# Autodesk Inventor assembly: Bed Arm Back for 4040 - Assembly
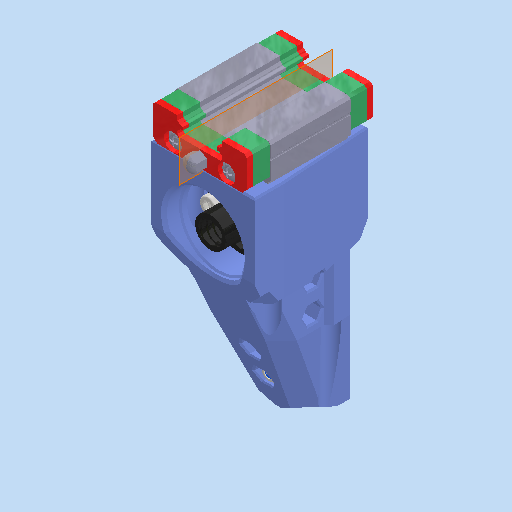
[picture p0: Inventor's stored thumbnail of the model, 512x512]
Saved by Autodesk Inventor 2023.2 (Build 272271000, 271)
## iProperties
Created: 2023-11-27
Part Number: Bed Arm Back for 4040 - Assembly
Document SubType Name: Assembly
Designer: Nils Bade
Author: Nils Bade
## Documents named in this file (11)
- C:\Users\nilsb\Documents\Inventor\Projektarbeit-Bade\RatRig_Bade\Bed Arm Back for 4040 - Assembly.iam
- C:\Users\nilsb\Documents\Inventor\Projektarbeit-Bade\RatRig_modified\Bed Arm Back for 4040.ipt
- C:\Users\nilsb\Documents\Inventor\Projektarbeit-Bade\RatRig_modified\MGN15 Linear-Rail-Block.ipt
- C:\Users\nilsb\Documents\Inventor\Projektarbeit-Bade\Schrauben\Cap Head Screw M3x12 v2.ipt
- C:\Users\nilsb\Documents\Inventor\Projektarbeit-Bade\Schrauben\Cap Head Screw M3x8 v2.ipt
- C:\Users\nilsb\Documents\Inventor\Projektarbeit-Bade\RatRig_Standards\Leadscrew Nut - POM - TR8_4 v1.ipt
- C:\Users\nilsb\Documents\Inventor\Projektarbeit-Bade\RatRig_Standards\Rat Rig Bi-Material Lead Screw Decoupler v1.ipt
- C:\Users\nilsb\Documents\Inventor\Projektarbeit-Bade\RatRig_Standards\Magnet - 20x10x5mm - Two hole (M3 Countersink screws) v1.ipt
- C:\Users\nilsb\Documents\Inventor\Projektarbeit-Bade\RatRig_Standards\Dowel Pin - 3x35mm v1.ipt
- C:\Users\nilsb\Documents\Inventor\Projektarbeit-Bade\RatRig_Standards\Hex Locking Nut - M3 v2.ipt
- C:\Users\nilsb\Documents\Inventor\Projektarbeit-Bade\Schrauben\Countersink Screw M3x12 v2.ipt
## Components (19 placed, 10 different names)
1. Bed Arm Back for 4040:1 — Passend:1, Passend:2, Passend:3, Passend:4, Passend:5, Passend:6, Passend:7, Passend:8, Passend:9, Passend:10, Passend:11, Passend:12, Passend:13, Passend:14, Passend:15, Passend:16, Passend:19, Passend:27, Passend:28, Passend:29, Passend:34, Passend:35, Passend:38, Passend:39, Winkel:1, Winkel:2, Passend:40, Passend:41
2. MGN15 Linear-Rail-Block:1 — Passend:1, Passend:2, Passend:3
3. Cap Head Screw M3x12 v2:1 — Passend:4, Passend:8
4. Cap Head Screw M3x12 v2:2 — Passend:6, Passend:11
5. Cap Head Screw M3x12 v2:3 — Passend:5, Passend:9
6. Cap Head Screw M3x12 v2:4 — Passend:7, Passend:10
7. Cap Head Screw M3x8 v2:1 — Passend:24, Passend:25
8. Cap Head Screw M3x8 v2:2 — Passend:23, Passend:26
9. Cap Head Screw M3x8 v2:3 — Passend:14, Passend:16, Passend:17
10. Cap Head Screw M3x8 v2:4 — Passend:13, Passend:15, Passend:18
11. Leadscrew Nut - POM - TR8_4 v1:1 — Passend:20, Passend:21, Passend:22, Passend:25, Passend:26
12. Rat Rig Bi-Material Lead Screw Decoupler v1:1 — Passend:12, Passend:17, Passend:18, Passend:19, Passend:20, Passend:21, Passend:22, Passend:23, Passend:24
13. Magnet - 20x10x5mm - Two hole (M3 Countersink screws) v1:1 — Passend:27, Passend:28, Passend:29, Passend:30, Passend:31, Passend:32, Passend:33
14. Dowel Pin - 3x35mm v1:1 — Passend:35, Passend:38
15. Dowel Pin - 3x35mm v1:2 — Passend:34, Passend:39
16. Hex Locking Nut - M3 v2:1 — Passend:36, Winkel:2, Passend:41
17. Hex Locking Nut - M3 v2:2 — Passend:37, Winkel:1, Passend:40
18. Countersink Screw M3x12 v2:1 — Passend:31, Passend:33, Passend:37
19. Countersink Screw M3x12 v2:2 — Passend:30, Passend:32, Passend:36
## Relationships (43: Mate 41, Angle 2)
- Passend:1 [Mate]: Bed Arm Back for 4040:1 ↔ MGN15 Linear-Rail-Block:1
- Passend:2 [Mate]: Bed Arm Back for 4040:1 ↔ MGN15 Linear-Rail-Block:1
- Passend:3 [Mate]: Bed Arm Back for 4040:1 ↔ MGN15 Linear-Rail-Block:1
- Passend:4 [Mate]: Bed Arm Back for 4040:1 ↔ Cap Head Screw M3x12 v2:1
- Passend:5 [Mate]: Bed Arm Back for 4040:1 ↔ Cap Head Screw M3x12 v2:3
- Passend:6 [Mate]: Bed Arm Back for 4040:1 ↔ Cap Head Screw M3x12 v2:2
- Passend:7 [Mate]: Bed Arm Back for 4040:1 ↔ Cap Head Screw M3x12 v2:4
- Passend:8 [Mate]: Bed Arm Back for 4040:1 ↔ Cap Head Screw M3x12 v2:1
- Passend:9 [Mate]: Bed Arm Back for 4040:1 ↔ Cap Head Screw M3x12 v2:3
- Passend:10 [Mate]: Bed Arm Back for 4040:1 ↔ Cap Head Screw M3x12 v2:4
- Passend:11 [Mate]: Bed Arm Back for 4040:1 ↔ Cap Head Screw M3x12 v2:2
- Passend:12 [Mate]: Bed Arm Back for 4040:1 ↔ Rat Rig Bi-Material Lead Screw Decoupler v1:1
- Passend:13 [Mate]: Bed Arm Back for 4040:1 ↔ Cap Head Screw M3x8 v2:4
- Passend:14 [Mate]: Bed Arm Back for 4040:1 ↔ Cap Head Screw M3x8 v2:3
- Passend:15 [Mate]: Bed Arm Back for 4040:1 ↔ Cap Head Screw M3x8 v2:4
- Passend:16 [Mate]: Bed Arm Back for 4040:1 ↔ Cap Head Screw M3x8 v2:3
- Passend:17 [Mate]: Cap Head Screw M3x8 v2:3 ↔ Rat Rig Bi-Material Lead Screw Decoupler v1:1
- Passend:18 [Mate]: Cap Head Screw M3x8 v2:4 ↔ Rat Rig Bi-Material Lead Screw Decoupler v1:1
- Passend:19 [Mate]: Bed Arm Back for 4040:1 ↔ Rat Rig Bi-Material Lead Screw Decoupler v1:1
- Passend:20 [Mate]: Leadscrew Nut - POM - TR8_4 v1:1 ↔ Rat Rig Bi-Material Lead Screw Decoupler v1:1
- Passend:21 [Mate]: Leadscrew Nut - POM - TR8_4 v1:1 ↔ Rat Rig Bi-Material Lead Screw Decoupler v1:1
- Passend:22 [Mate]: Leadscrew Nut - POM - TR8_4 v1:1 ↔ Rat Rig Bi-Material Lead Screw Decoupler v1:1
- Passend:23 [Mate]: Cap Head Screw M3x8 v2:2 ↔ Rat Rig Bi-Material Lead Screw Decoupler v1:1
- Passend:24 [Mate]: Cap Head Screw M3x8 v2:1 ↔ Rat Rig Bi-Material Lead Screw Decoupler v1:1
- Passend:25 [Mate]: Cap Head Screw M3x8 v2:1 ↔ Leadscrew Nut - POM - TR8_4 v1:1
- Passend:26 [Mate]: Cap Head Screw M3x8 v2:2 ↔ Leadscrew Nut - POM - TR8_4 v1:1
- Passend:27 [Mate]: Bed Arm Back for 4040:1 ↔ Magnet - 20x10x5mm - Two hole (M3 Countersink screws) v1:1
- Passend:28 [Mate]: Bed Arm Back for 4040:1 ↔ Magnet - 20x10x5mm - Two hole (M3 Countersink screws) v1:1
- Passend:29 [Mate]: Bed Arm Back for 4040:1 ↔ Magnet - 20x10x5mm - Two hole (M3 Countersink screws) v1:1
- Passend:30 [Mate]: Magnet - 20x10x5mm - Two hole (M3 Countersink screws) v1:1 ↔ Countersink Screw M3x12 v2:2
- Passend:31 [Mate]: Magnet - 20x10x5mm - Two hole (M3 Countersink screws) v1:1 ↔ Countersink Screw M3x12 v2:1
- Passend:32 [Mate]: Magnet - 20x10x5mm - Two hole (M3 Countersink screws) v1:1 ↔ Countersink Screw M3x12 v2:2
- Passend:33 [Mate]: Magnet - 20x10x5mm - Two hole (M3 Countersink screws) v1:1 ↔ Countersink Screw M3x12 v2:1
- Passend:34 [Mate]: Bed Arm Back for 4040:1 ↔ Dowel Pin - 3x35mm v1:2
- Passend:35 [Mate]: Bed Arm Back for 4040:1 ↔ Dowel Pin - 3x35mm v1:1
- Passend:36 [Mate]: Hex Locking Nut - M3 v2:1 ↔ Countersink Screw M3x12 v2:2
- Passend:37 [Mate]: Hex Locking Nut - M3 v2:2 ↔ Countersink Screw M3x12 v2:1
- Passend:38 [Mate]: Bed Arm Back for 4040:1 ↔ Dowel Pin - 3x35mm v1:1
- Passend:39 [Mate]: Bed Arm Back for 4040:1 ↔ Dowel Pin - 3x35mm v1:2
- Winkel:1 [Angle] (0 deg): Bed Arm Back for 4040:1 ↔ Hex Locking Nut - M3 v2:2
- Winkel:2 [Angle] (0 deg): Bed Arm Back for 4040:1 ↔ Hex Locking Nut - M3 v2:1
- Passend:40 [Mate]: Bed Arm Back for 4040:1 ↔ Hex Locking Nut - M3 v2:2
- Passend:41 [Mate]: Bed Arm Back for 4040:1 ↔ Hex Locking Nut - M3 v2:1
